# Autodesk Inventor assembly: Propeller
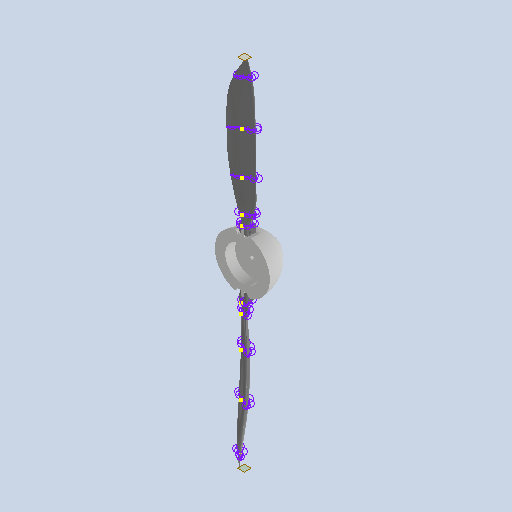
[picture p0: Inventor's stored thumbnail of the model, 512x512]
Saved by Autodesk Inventor 2023.4 (Build 274418000, 418)
## iProperties
Created: 2021-05-01
Part Number: Propeller
Document SubType Name: Assembly
Designer: armin
Author: armin
## Documents named in this file (3)
- C:\Users\Malthe Sennels\OneDrive - Aalborg Universitet\Inventor 3D filer\Flyver\Propeller.iam
- C:\Users\Malthe Sennels\OneDrive - Aalborg Universitet\Inventor 3D filer\Flyver\Prop center.ipt
- C:\Users\Malthe Sennels\OneDrive - Aalborg Universitet\Inventor 3D filer\Flyver\Prop.ipt
## Components (3 placed, 2 different names)
1. Prop center:1 — Mate:1, Mate:2, Mate:3, Mate:4, Mate:5, Mate:6
2. Prop:1 — Mate:1, Mate:2, Mate:5
3. Prop:2 — Mate:3, Mate:4, Mate:6
## Relationships (6: Mate 6)
- Mate:1: Prop center:1 ↔ Prop:1
- Mate:2: Prop center:1 ↔ Prop:1
- Mate:3: Prop center:1 ↔ Prop:2
- Mate:4: Prop center:1 ↔ Prop:2
- Mate:5: Prop center:1 ↔ Prop:1
- Mate:6: Prop center:1 ↔ Prop:2
